# Autodesk Inventor assembly: foiurbar
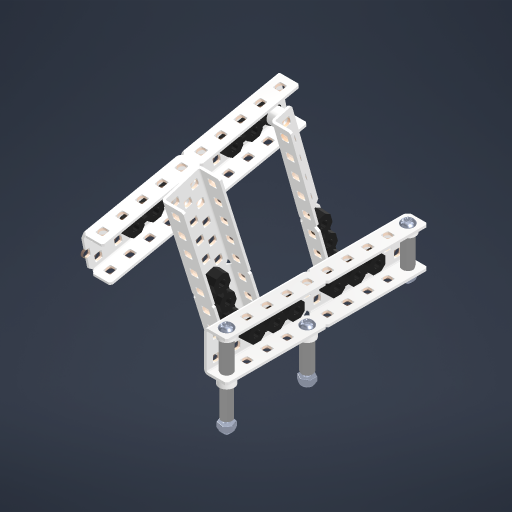
[picture p0: Inventor's stored thumbnail of the model, 512x512]
Saved by Autodesk Inventor 2023 (Build 270158000, 158)
## iProperties
Created: 2023-08-08
Part Number: foiurbar
Document SubType Name: Assembly
Designer: srbel
Author: srbel
## Documents named in this file (14)
- C:\CAD\OverUnderCAD\Drive\foiurbar.iam
- C:\CAD\OverUnderCAD\VEX-CAD-Inventor-1.4.0\Structure\C Channel\Aluminum 1x2x1\Alu C 1x2x1x10.ipt
- C:\CAD\OverUnderCAD\VEX-CAD-Inventor-1.4.0\Motion\Spacers\Spacer Nylon .313 OD\NSpacer .313 OD x .125.ipt
- C:\CAD\OverUnderCAD\VEX-CAD-Inventor-1.4.0\Motion\Spacers\Spacer Nylon .313 OD.ipt
- C:\CAD\OverUnderCAD\VEX-CAD-Inventor-1.4.0\Structure\Standoff\Standoff .75.ipt
- C:\CAD\OverUnderCAD\VEX-CAD-Inventor-1.4.0\Structure\Standoff.ipt
- C:\CAD\OverUnderCAD\VEX-CAD-Inventor-1.4.0\Structure\Hardware\Screw Steel - Star\SScrew Star Threaded 2.250.ipt
- C:\CAD\OverUnderCAD\VEX-CAD-Inventor-1.4.0\Structure\Hardware\Screw Steel - Star.ipt
- C:\CAD\OverUnderCAD\VEX-CAD-Inventor-1.4.0\Structure\Hardware\Nut Thin Nylock.ipt
- C:\CAD\OverUnderCAD\VEX-CAD-Inventor-1.4.0\Structure\Hardware\Screw Steel - Star\SScrew Star Threaded 1.250.ipt
- C:\CAD\OverUnderCAD\VEX-CAD-Inventor-1.4.0\Motion\Shaft LS\Bearing Flat.ipt
- C:\CAD\OverUnderCAD\VEX-CAD-Inventor-1.4.0\Structure\Angle\Aluminum\1x1\Alu Angle 1x1x8.ipt
- C:\CAD\OverUnderCAD\VEX-CAD-Inventor-1.4.0\Structure\C Channel\Aluminum 1x2x1\Alu C 1x2x1x8.ipt
- C:\CAD\OverUnderCAD\VEX-CAD-Inventor-1.4.0\Motion\Spacers\Spacer Nylon .313 OD\NSpacer .313 OD x .250.ipt
## Components (28 placed, 10 different names)
1. Alu C 1x2x1x10:1 — Insert:16, Insert:17, Insert:18, Insert:19, Insert:20, Insert:62, Insert:63
2. NSpacer .313 OD x .125:1
3. Standoff .75:1
4. NSpacer .313 OD x .125:2
5. Standoff .75:2
6. Standoff .75:3 — Insert:15
7. NSpacer .313 OD x .125:3
8. Standoff .75:4
9. SScrew Star Threaded 2.250:1
10. Nut Thin Nylock:1
11. Nut Thin Nylock:2
12. Nut Thin Nylock:3
13. SScrew Star Threaded 1.250:2
14. NSpacer .313 OD x .125:5 — Insert:15, Insert:16
15. Bearing Flat:1 — Insert:17, Insert:18
16. Bearing Flat:2 — Insert:19
17. SScrew Star Threaded 1.250:3 — Insert:20
18. Bearing Flat:5 — Insert:54, Insert:55, Insert:60
19. Bearing Flat:6 — Insert:52, Insert:53, Insert:61
20. Alu Angle 1x1x8:1 — Insert:52, Insert:53, Insert:65
21. Alu C 1x2x1x8:1 — Insert:54, Insert:55, Insert:69
22. Alu C 1x2x1x10:2 — Insert:56, Insert:57, Insert:67, Insert:68
23. Bearing Flat:7 — Insert:56, Insert:57, Insert:64
24. NSpacer .313 OD x .250:19 — Insert:60, Insert:62
25. NSpacer .313 OD x .250:20 — Insert:61, Insert:63
26. NSpacer .313 OD x .250:21 — Insert:64, Insert:65
27. Bearing Flat:8 — Insert:67, Insert:68
28. NSpacer .313 OD x .250:22 — Insert:69
## Relationships (33: Insert 33)
- [Insert]: NSpacer .313 OD x .125:1 ↔ Standoff .75:1
- [Insert]: Alu C 1x2x1x10:1 ↔ NSpacer .313 OD x .125:1
- [Insert]: NSpacer .313 OD x .125:2 ↔ Standoff .75:2
- [Insert]: Alu C 1x2x1x10:1 ↔ NSpacer .313 OD x .125:2
- [Insert]: NSpacer .313 OD x .125:3 ↔ Standoff .75:4
- [Insert] (1.5875 mm): Alu C 1x2x1x10:1 ↔ NSpacer .313 OD x .125:3
- [Insert]: Alu C 1x2x1x10:1 ↔ SScrew Star Threaded 2.250:1
- [Insert] (1.5875 mm): Standoff .75:3 ↔ Nut Thin Nylock:2
- [Insert] (1.5875 mm): Standoff .75:4 ↔ Nut Thin Nylock:1
- [Insert]: Alu C 1x2x1x10:1 ↔ Nut Thin Nylock:3
- [Insert]: Alu C 1x2x1x10:1 ↔ SScrew Star Threaded 1.250:2
- Insert:15: Standoff .75:3 ↔ NSpacer .313 OD x .125:5
- Insert:16 (1.5875 mm): Alu C 1x2x1x10:1 ↔ NSpacer .313 OD x .125:5
- Insert:17: Alu C 1x2x1x10:1 ↔ Bearing Flat:1
- Insert:18: Alu C 1x2x1x10:1 ↔ Bearing Flat:1
- Insert:19: Alu C 1x2x1x10:1 ↔ Bearing Flat:2
- Insert:20: Alu C 1x2x1x10:1 ↔ SScrew Star Threaded 1.250:3
- Insert:52: Bearing Flat:6 ↔ Alu Angle 1x1x8:1
- Insert:53: Bearing Flat:6 ↔ Alu Angle 1x1x8:1
- Insert:54: Bearing Flat:5 ↔ Alu C 1x2x1x8:1
- Insert:55: Bearing Flat:5 ↔ Alu C 1x2x1x8:1
- Insert:56: Alu C 1x2x1x10:2 ↔ Bearing Flat:7
- Insert:57: Alu C 1x2x1x10:2 ↔ Bearing Flat:7
- Insert:60: Bearing Flat:5 ↔ NSpacer .313 OD x .250:19
- Insert:61: Bearing Flat:6 ↔ NSpacer .313 OD x .250:20
- Insert:62: Alu C 1x2x1x10:1 ↔ NSpacer .313 OD x .250:19
- Insert:63: Alu C 1x2x1x10:1 ↔ NSpacer .313 OD x .250:20
- Insert:64: Bearing Flat:7 ↔ NSpacer .313 OD x .250:21
- Insert:65: Alu Angle 1x1x8:1 ↔ NSpacer .313 OD x .250:21
- [Insert]: Bearing Flat:8 ↔ NSpacer .313 OD x .250:22
- Insert:67: Alu C 1x2x1x10:2 ↔ Bearing Flat:8
- Insert:68: Alu C 1x2x1x10:2 ↔ Bearing Flat:8
- Insert:69: Alu C 1x2x1x8:1 ↔ NSpacer .313 OD x .250:22
## Named parameters: d288_d1 = 0 mm, d290_d1 = 0 mm, d294_d292_d1 = 0 mm, d75_d73 = 0 mm
